# Autodesk Inventor assembly: Weight assembly
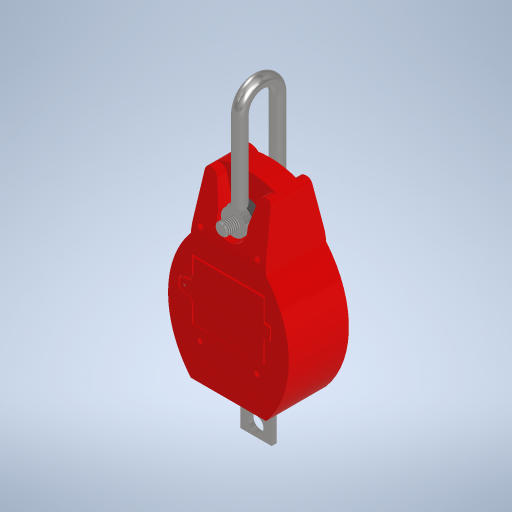
[picture p0: Inventor's stored thumbnail of the model, 512x512]
Saved by Autodesk Inventor 2023 (Build 270158000, 158)
## iProperties
Created: 2023-12-11
Part Number: Weight assembly
Document SubType Name: Assembly
Designer: User
Author: User
## Documents named in this file (13)
- G:\Downloads\INVENTOR WEIGH SCALE\Weight assembly.iam
- G:\Downloads\INVENTOR WEIGH SCALE\Back.ipt
- G:\Downloads\INVENTOR WEIGH SCALE\Battery holder.ipt
- G:\Downloads\SOLIDWORKS (1)\loadcelloriginal1.ipt
- G:\Downloads\INVENTOR WEIGH SCALE\Front.ipt
- G:\Downloads\INVENTOR WEIGH SCALE\Rubber ring.ipt
- G:\Downloads\INVENTOR WEIGH SCALE\Hook.ipt
- G:\Documents\Inventor\Content Center Files\R2023\en-US\AS 1427(01)\AS 1427 - M10 x 50(3).ipt
- G:\Downloads\INVENTOR WEIGH SCALE\Battery holder lid.ipt
- G:\Downloads\INVENTOR WEIGH SCALE\Limit switch.iam
- C:\Users\User\Downloads\Compressed\az-delivery-1-8-inch-tft-display-spi-1.snapshot.6\AZ-Delivery 1.8 inch TFT Display SPI.ipt
- G:\Downloads\tft esp32  indicator v4.ipt
- G:\Downloads\INVENTOR WEIGH SCALE\Hook-Extension.ipt
## Components (13 placed, 12 different names)
1. Back:1 — Mate:1, Mate:2, Mate:4, Mate:5, Mate:6, Mate:9, Flush:2, Flush:5, Mate:39
2. Battery holder:1 — Mate:1, Mate:2, Mate:23
3. loadcelloriginal1:1 — Mate:4, Mate:5, Mate:8, Mate:10, Mate:37, Mate:38
4. Front:1 — Mate:6, Mate:24, Mate:25, Mate:26, Mate:29, Mate:33, Mate:34, Flush:4, Flush:5, Mate:39
5. Rubber ring:1 — Mate:8, Mate:19, Mate:20
6. Rubber ring:2 — Mate:9, Mate:10
7. Hook:1 — Mate:19, Mate:20, Mate:21, Mate:22
8. AS 1427 - Metric M10 x 50:1 — Mate:21, Mate:22
9. Battery holder lid:1 — Mate:23, Flush:2
10. Limit switch:1 [sub-assembly] — Mate:24, Mate:25, Mate:26
11. AZ-Delivery 1.8 inch TFT Display SPI:1 — Flush:3, Flush:4
12. tft esp32  indicator v4:1 — Flush:3, Mate:29, Mate:33, Mate:34
13. Hook-Extension:1 — Mate:37, Mate:38
## Relationships (26: Mate 22, Flush 4)
- Mate:1: Back:1 ↔ Battery holder:1
- Mate:2: Back:1 ↔ Battery holder:1
- Mate:4: Back:1 ↔ loadcelloriginal1:1
- Mate:5: Back:1 ↔ loadcelloriginal1:1
- Mate:6: Back:1 ↔ Front:1
- Mate:8: loadcelloriginal1:1 ↔ Rubber ring:1
- Mate:9: Back:1 ↔ Rubber ring:2
- Mate:10 (1 mm): loadcelloriginal1:1 ↔ Rubber ring:2
- Mate:19: Rubber ring:1 ↔ Hook:1
- Mate:20 (4 mm): Rubber ring:1 ↔ Hook:1
- Mate:21: Hook:1 ↔ AS 1427 - Metric M10 x 50:1
- Mate:22: Hook:1 ↔ AS 1427 - Metric M10 x 50:1
- Mate:23: Battery holder:1 ↔ Battery holder lid:1
- Flush:2: Back:1 ↔ Battery holder lid:1
- Mate:24: Front:1 ↔ Limit switch:1
- Mate:25 (0.5 mm): Front:1 ↔ Limit switch:1
- Mate:26: Front:1 ↔ Limit switch:1
- Flush:3 (8.128 mm): AZ-Delivery 1.8 inch TFT Display SPI:1 ↔ tft esp32  indicator v4:1
- Mate:29: Front:1 ↔ tft esp32  indicator v4:1
- Mate:33: Front:1 ↔ tft esp32  indicator v4:1
- Mate:34: Front:1 ↔ tft esp32  indicator v4:1
- Flush:4 (1 mm): Front:1 ↔ AZ-Delivery 1.8 inch TFT Display SPI:1
- Mate:37: loadcelloriginal1:1 ↔ Hook-Extension:1
- Mate:38: loadcelloriginal1:1 ↔ Hook-Extension:1
- Flush:5: Back:1 ↔ Front:1
- Mate:39: Back:1 ↔ Front:1
